# Autodesk Inventor assembly: BREEZE-S02
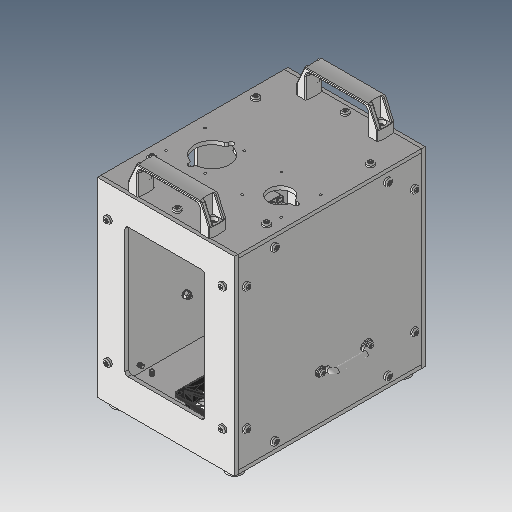
[picture p0: Inventor's stored thumbnail of the model, 512x512]
Saved by Autodesk Inventor 2020 (Build 240168000, 168)
## iProperties
Created: 2020-04-12
Part Number: BREEZE-S02
Document SubType Name: Assembly
Designer: John K
Description: PANEL ASSEMBLY
Author: John K
## Documents named in this file (22)
- C:\GrabCAD\MTL Ventilator Design\BREEZE\Subassemblies\BREEZE-S02.iam
- C:\GrabCAD\MTL Ventilator Design\BREEZE\Manufactured Parts\BREEZE-M05.ipt
- C:\GrabCAD\MTL Ventilator Design\BREEZE\Manufactured Parts\BREEZE-M10.ipt
- C:\GrabCAD\MTL Ventilator Design\BREEZE\Manufactured Parts\BREEZE-M06.ipt
- C:\GrabCAD\MTL Ventilator Design\BREEZE\Manufactured Parts\BREEZE-M07.ipt
- C:\GrabCAD\MTL Ventilator Design\BREEZE\Manufactured Parts\BREEZE-M08.ipt
- C:\GrabCAD\MTL Ventilator Design\BREEZE\Manufactured Parts\BREEZE-M09.ipt
- C:\GrabCAD\MTL Ventilator Design\BREEZE\Commercial Parts\McMaster\M5x10mm Nylon Screw.ipt
- C:\GrabCAD\MTL Ventilator Design\BREEZE\Commercial Parts\McMaster\Foot.ipt
- C:\GrabCAD\MTL Ventilator Design\BREEZE\Commercial Parts\McMaster\M4x16mm Nylon Screw.ipt
- C:\GrabCAD\MTL Ventilator Design\BREEZE\Commercial Parts\McMaster\M4 Nylon Washer.ipt
- C:\GrabCAD\MTL Ventilator Design\BREEZE\Commercial Parts\McMaster\M4 Locknut.ipt
- C:\GrabCAD\MTL Ventilator Design\BREEZE\Commercial Parts\McMaster\Handle.ipt
- C:\GrabCAD\MTL Ventilator Design\BREEZE\Commercial Parts\McMaster\M5x16mm Nylon Screw.ipt
- C:\GrabCAD\MTL Ventilator Design\BREEZE\Commercial Parts\McMaster\Webbing Guide.ipt
- C:\GrabCAD\MTL Ventilator Design\BREEZE\Commercial Parts\Electronics\Toggle Switch.ipt
- C:\GrabCAD\MTL Ventilator Design\BREEZE\Commercial Parts\Electronics\Switch Cover.ipt
- C:\GrabCAD\MTL Ventilator Design\BREEZE\Commercial Parts\Electronics\Power Connector.ipt
- C:\GrabCAD\MTL Ventilator Design\BREEZE\Commercial Parts\McMaster\M3 Nylon Washer.ipt
- C:\GrabCAD\MTL Ventilator Design\BREEZE\Commercial Parts\McMaster\M3 Locknut.ipt
- C:\GrabCAD\MTL Ventilator Design\BREEZE\Commercial Parts\McMaster\M3x16mm Nylon Screw.ipt
- C:\GrabCAD\MTL Ventilator Design\BREEZE\Commercial Parts\Electronics\Chassis Fan.ipt
## Components (103 placed, 21 different names)
1. BREEZE-M05:1 — Mate:1, Flush:1, Flush:2, Flush:3, Symmetry:1, Mate:4, Insert:23, Insert:24, Insert:25, Insert:26, Insert:27, Insert:28, Insert:40, Insert:41, Insert:42, Insert:43, Insert:48, Insert:49, Insert:50, Insert:51, Mate:16, Mate:17, Mate:18, Insert:92, Insert:93, Insert:94, Insert:95
2. BREEZE-M06:1 — Flush:4, Mate:2, Flush:5, Flush:6, Mate:3, Insert:1, Insert:2, Insert:3, Insert:4
3. BREEZE-M07:1 — Flush:6, Mate:3, Mate:4, Mate:5, Flush:7, Insert:5, Insert:6, Insert:7, Insert:8, Insert:9, Insert:10, Insert:11, Insert:29, Insert:65, Mate:12, Insert:70, Insert:71
4. BREEZE-M08:1 — Flush:7, Flush:8, Mate:6, Mate:8, Flush:9, Insert:12, Insert:13, Insert:14, Insert:15, Insert:37, Insert:38, Insert:39, Angle:1, Angle:2
5. BREEZE-M09:1 — Mate:7, Mate:8, Flush:9, Insert:16, Insert:17, Insert:18, Insert:19, Insert:20, Insert:21, Insert:22, Insert:36, Insert:62, Mate:11, Insert:68, Insert:69, Insert:76, Insert:77, Mate:13, Mate:14, Mate:15, Insert:78, Insert:79
6. BREEZE-M10:1 — Flush:2, Flush:3, Symmetry:1, Flush:4, Mate:2, Flush:5, Mate:5, Flush:8, Mate:6, Mate:7, Insert:30, Insert:31, Insert:32, Insert:33, Insert:34, Insert:35, Insert:56, Insert:57, Mate:9, Mate:10
7. Foot:1 — Insert:40
8. Foot:2 — Insert:41
9. Foot:3 — Insert:42
10. Foot:4 — Insert:43
11. Handle:1 — Insert:56, Mate:9
12. Handle:2 — Insert:57, Mate:10
13. Webbing Guide:1 — Insert:62, Mate:11, Insert:63, Insert:64
14. Webbing Guide:2 — Insert:65, Mate:12, Insert:66, Insert:67
15. Power Connector:1 — Mate:13, Mate:14, Mate:15, Insert:82, Insert:83
16. Toggle Switch:1 — Insert:76, Angle:1
17. Switch Cover:1 — Insert:77, Angle:2
18. Chassis Fan:1 — Mate:16, Mate:17, Mate:18, Insert:84, Insert:85, Insert:86, Insert:87
19. M4 Nylon Washer:9 — Insert:84, Insert:91
20. M4 Nylon Washer:10 — Insert:85, Insert:90
21. M4 Nylon Washer:11 — Insert:86, Insert:88
22. M4 Nylon Washer:12 — Insert:87, Insert:89
23. M4 Locknut:9 — Insert:88
24. M4 Locknut:10 — Insert:89
25. M4 Locknut:11 — Insert:90
26. M4 Locknut:12 — Insert:91
27. M4x16mm Nylon Screw:9 — Insert:92
28. M4x16mm Nylon Screw:10 — Insert:93
29. M4x16mm Nylon Screw:11 — Insert:94
30. M4x16mm Nylon Screw:12 — Insert:95
31. M3 Nylon Washer:1 — Insert:78, Insert:80
32. M3 Nylon Washer:2 — Insert:79, Insert:81
33. M3 Locknut:1 — Insert:80
34. M3 Locknut:2 — Insert:81
35. M3x16mm Nylon Screw:1 — Insert:82
36. M3x16mm Nylon Screw:2 — Insert:83
37. M4x16mm Nylon Screw:7 — Insert:66
38. M4x16mm Nylon Screw:8 — Insert:67
39. M4 Nylon Washer:5 — Insert:68, Insert:72
40. M4 Nylon Washer:6 — Insert:69, Insert:73
41. M4 Nylon Washer:7 — Insert:70, Insert:74
42. M4 Nylon Washer:8 — Insert:71, Insert:75
43. M4 Locknut:5 — Insert:72
44. M4 Locknut:6 — Insert:73
45. M4 Locknut:7 — Insert:74
46. M4 Locknut:8 — Insert:75
47. M4x16mm Nylon Screw:5 — Insert:63
48. M4x16mm Nylon Screw:6 — Insert:64
49. M5x16mm Nylon Screw:1
50. M5x16mm Nylon Screw:2
51. M5x16mm Nylon Screw:4
52. M5x16mm Nylon Screw:3
53. M4x16mm Nylon Screw:1
54. M4x16mm Nylon Screw:2
55. M4x16mm Nylon Screw:3
56. M4x16mm Nylon Screw:4
57. M4 Nylon Washer:1 — Insert:48, Insert:52
58. M4 Nylon Washer:2 — Insert:49, Insert:53
59. M4 Nylon Washer:3 — Insert:50, Insert:54
60. M4 Nylon Washer:4 — Insert:51, Insert:55
61. M4 Locknut:1 — Insert:52
62. M4 Locknut:2 — Insert:53
63. M4 Locknut:3 — Insert:54
64. M4 Locknut:4 — Insert:55
65. M5x10mm Nylon Screw:1 — Insert:1
66. M5x10mm Nylon Screw:2 — Insert:2
67. M5x10mm Nylon Screw:3 — Insert:3
68. M5x10mm Nylon Screw:4 — Insert:4
69. M5x10mm Nylon Screw:5 — Insert:5
70. M5x10mm Nylon Screw:6 — Insert:6
71. M5x10mm Nylon Screw:7 — Insert:7
72. M5x10mm Nylon Screw:8 — Insert:8
73. M5x10mm Nylon Screw:9 — Insert:9
74. M5x10mm Nylon Screw:10 — Insert:10
75. M5x10mm Nylon Screw:11 — Insert:11
76. M5x10mm Nylon Screw:12 — Insert:12
77. M5x10mm Nylon Screw:13 — Insert:13
78. M5x10mm Nylon Screw:14 — Insert:14
79. M5x10mm Nylon Screw:15 — Insert:15
80. M5x10mm Nylon Screw:16 — Insert:16
81. M5x10mm Nylon Screw:17 — Insert:17
82. M5x10mm Nylon Screw:18 — Insert:18
83. M5x10mm Nylon Screw:19 — Insert:19
84. M5x10mm Nylon Screw:20 — Insert:20
85. M5x10mm Nylon Screw:21 — Insert:21
86. M5x10mm Nylon Screw:22 — Insert:22
87. M5x10mm Nylon Screw:23 — Insert:23
88. M5x10mm Nylon Screw:24 — Insert:24
89. M5x10mm Nylon Screw:25 — Insert:25
90. M5x10mm Nylon Screw:26 — Insert:26
91. M5x10mm Nylon Screw:27 — Insert:27
92. M5x10mm Nylon Screw:28 — Insert:28
93. M5x10mm Nylon Screw:29 — Insert:29
94. M5x10mm Nylon Screw:30 — Insert:30
95. M5x10mm Nylon Screw:31 — Insert:31
96. M5x10mm Nylon Screw:32 — Insert:32
97. M5x10mm Nylon Screw:33 — Insert:33
98. M5x10mm Nylon Screw:34 — Insert:34
99. M5x10mm Nylon Screw:35 — Insert:35
100. M5x10mm Nylon Screw:36 — Insert:36
101. M5x10mm Nylon Screw:37 — Insert:37
102. M5x10mm Nylon Screw:38 — Insert:38
103. M5x10mm Nylon Screw:39 — Insert:39
## Relationships (125: Insert 95, Mate 18, Flush 9, Angle 2, Symmetry 1)
- Mate:1: BREEZE-M05:1
- Flush:1: BREEZE-M05:1
- Flush:2: BREEZE-M05:1 ↔ BREEZE-M10:1
- Flush:3: BREEZE-M05:1 ↔ BREEZE-M10:1
- Symmetry:1: BREEZE-M05:1 ↔ BREEZE-M10:1
- Flush:4: BREEZE-M06:1 ↔ BREEZE-M10:1
- Mate:2: BREEZE-M06:1 ↔ BREEZE-M10:1
- Flush:5: BREEZE-M06:1 ↔ BREEZE-M10:1
- Flush:6: BREEZE-M06:1 ↔ BREEZE-M07:1
- Mate:3: BREEZE-M06:1 ↔ BREEZE-M07:1
- Mate:4: BREEZE-M05:1 ↔ BREEZE-M07:1
- Mate:5: BREEZE-M07:1 ↔ BREEZE-M10:1
- Flush:7: BREEZE-M07:1 ↔ BREEZE-M08:1
- Flush:8: BREEZE-M08:1 ↔ BREEZE-M10:1
- Mate:6: BREEZE-M08:1 ↔ BREEZE-M10:1
- Mate:7: BREEZE-M09:1 ↔ BREEZE-M10:1
- Mate:8: BREEZE-M08:1 ↔ BREEZE-M09:1
- Flush:9: BREEZE-M08:1 ↔ BREEZE-M09:1
- Insert:1: BREEZE-M06:1 ↔ M5x10mm Nylon Screw:1
- Insert:2: BREEZE-M06:1 ↔ M5x10mm Nylon Screw:2
- Insert:3: BREEZE-M06:1 ↔ M5x10mm Nylon Screw:3
- Insert:4: BREEZE-M06:1 ↔ M5x10mm Nylon Screw:4
- Insert:5: BREEZE-M07:1 ↔ M5x10mm Nylon Screw:5
- Insert:6: BREEZE-M07:1 ↔ M5x10mm Nylon Screw:6
- Insert:7: BREEZE-M07:1 ↔ M5x10mm Nylon Screw:7
- Insert:8: BREEZE-M07:1 ↔ M5x10mm Nylon Screw:8
- Insert:9: BREEZE-M07:1 ↔ M5x10mm Nylon Screw:9
- Insert:10: BREEZE-M07:1 ↔ M5x10mm Nylon Screw:10
- Insert:11: BREEZE-M07:1 ↔ M5x10mm Nylon Screw:11
- Insert:12: BREEZE-M08:1 ↔ M5x10mm Nylon Screw:12
- Insert:13: BREEZE-M08:1 ↔ M5x10mm Nylon Screw:13
- Insert:14: BREEZE-M08:1 ↔ M5x10mm Nylon Screw:14
- Insert:15: BREEZE-M08:1 ↔ M5x10mm Nylon Screw:15
- Insert:16: BREEZE-M09:1 ↔ M5x10mm Nylon Screw:16
- Insert:17: BREEZE-M09:1 ↔ M5x10mm Nylon Screw:17
- Insert:18: BREEZE-M09:1 ↔ M5x10mm Nylon Screw:18
- Insert:19: BREEZE-M09:1 ↔ M5x10mm Nylon Screw:19
- Insert:20: BREEZE-M09:1 ↔ M5x10mm Nylon Screw:20
- Insert:21: BREEZE-M09:1 ↔ M5x10mm Nylon Screw:21
- Insert:22: BREEZE-M09:1 ↔ M5x10mm Nylon Screw:22
- Insert:23: BREEZE-M05:1 ↔ M5x10mm Nylon Screw:23
- Insert:24: BREEZE-M05:1 ↔ M5x10mm Nylon Screw:24
- Insert:25: BREEZE-M05:1 ↔ M5x10mm Nylon Screw:25
- Insert:26: BREEZE-M05:1 ↔ M5x10mm Nylon Screw:26
- Insert:27: BREEZE-M05:1 ↔ M5x10mm Nylon Screw:27
- Insert:28: BREEZE-M05:1 ↔ M5x10mm Nylon Screw:28
- Insert:29: BREEZE-M07:1 ↔ M5x10mm Nylon Screw:29
- Insert:30: BREEZE-M10:1 ↔ M5x10mm Nylon Screw:30
- Insert:31: BREEZE-M10:1 ↔ M5x10mm Nylon Screw:31
- Insert:32: BREEZE-M10:1 ↔ M5x10mm Nylon Screw:32
- Insert:33: BREEZE-M10:1 ↔ M5x10mm Nylon Screw:33
- Insert:34: BREEZE-M10:1 ↔ M5x10mm Nylon Screw:34
- Insert:35: BREEZE-M10:1 ↔ M5x10mm Nylon Screw:35
- Insert:36: BREEZE-M09:1 ↔ M5x10mm Nylon Screw:36
- Insert:37: BREEZE-M08:1 ↔ M5x10mm Nylon Screw:37
- Insert:38: BREEZE-M08:1 ↔ M5x10mm Nylon Screw:38
- Insert:39: BREEZE-M08:1 ↔ M5x10mm Nylon Screw:39
- Insert:40: BREEZE-M05:1 ↔ Foot:1
- Insert:41: BREEZE-M05:1 ↔ Foot:2
- Insert:42: BREEZE-M05:1 ↔ Foot:3
- Insert:43: BREEZE-M05:1 ↔ Foot:4
- [Insert]: Foot:4 ↔ M4x16mm Nylon Screw:1
- [Insert]: Foot:1 ↔ M4x16mm Nylon Screw:2
- [Insert]: Foot:2 ↔ M4x16mm Nylon Screw:3
- [Insert]: Foot:3 ↔ M4x16mm Nylon Screw:4
- Insert:48: BREEZE-M05:1 ↔ M4 Nylon Washer:1
- Insert:49: BREEZE-M05:1 ↔ M4 Nylon Washer:2
- Insert:50: BREEZE-M05:1 ↔ M4 Nylon Washer:3
- Insert:51: BREEZE-M05:1 ↔ M4 Nylon Washer:4
- Insert:52: M4 Nylon Washer:1 ↔ M4 Locknut:1
- Insert:53: M4 Nylon Washer:2 ↔ M4 Locknut:2
- Insert:54: M4 Nylon Washer:3 ↔ M4 Locknut:3
- Insert:55: M4 Nylon Washer:4 ↔ M4 Locknut:4
- Insert:56: BREEZE-M10:1 ↔ Handle:1
- Insert:57: BREEZE-M10:1 ↔ Handle:2
- Mate:9: BREEZE-M10:1 ↔ Handle:1
- Mate:10: BREEZE-M10:1 ↔ Handle:2
- [Insert]: Handle:2 ↔ M5x16mm Nylon Screw:1
- [Insert]: Handle:2 ↔ M5x16mm Nylon Screw:2
- [Insert]: Handle:1 ↔ M5x16mm Nylon Screw:4
- [Insert]: Handle:1 ↔ M5x16mm Nylon Screw:3
- Insert:62: BREEZE-M09:1 ↔ Webbing Guide:1
- Mate:11: BREEZE-M09:1 ↔ Webbing Guide:1
- Insert:63: Webbing Guide:1 ↔ M4x16mm Nylon Screw:5
- Insert:64: Webbing Guide:1 ↔ M4x16mm Nylon Screw:6
- Insert:65: BREEZE-M07:1 ↔ Webbing Guide:2
- Mate:12: BREEZE-M07:1 ↔ Webbing Guide:2
- Insert:66: Webbing Guide:2 ↔ M4x16mm Nylon Screw:7
- Insert:67: Webbing Guide:2 ↔ M4x16mm Nylon Screw:8
- Insert:68: BREEZE-M09:1 ↔ M4 Nylon Washer:5
- Insert:69: BREEZE-M09:1 ↔ M4 Nylon Washer:6
- Insert:70: BREEZE-M07:1 ↔ M4 Nylon Washer:7
- Insert:71: BREEZE-M07:1 ↔ M4 Nylon Washer:8
- Insert:72: M4 Nylon Washer:5 ↔ M4 Locknut:5
- Insert:73: M4 Nylon Washer:6 ↔ M4 Locknut:6
- Insert:74: M4 Nylon Washer:7 ↔ M4 Locknut:7
- Insert:75: M4 Nylon Washer:8 ↔ M4 Locknut:8
- Insert:76: BREEZE-M09:1 ↔ Toggle Switch:1
- Angle:1 (0 deg): BREEZE-M08:1 ↔ Toggle Switch:1
- Insert:77: BREEZE-M09:1 ↔ Switch Cover:1
- Angle:2 (0 deg): BREEZE-M08:1 ↔ Switch Cover:1
- Mate:13: BREEZE-M09:1 ↔ Power Connector:1
- Mate:14: BREEZE-M09:1 ↔ Power Connector:1
- Mate:15: BREEZE-M09:1 ↔ Power Connector:1
- Insert:78: BREEZE-M09:1 ↔ M3 Nylon Washer:1
- Insert:79: BREEZE-M09:1 ↔ M3 Nylon Washer:2
- Insert:80: M3 Nylon Washer:1 ↔ M3 Locknut:1
- Insert:81: M3 Nylon Washer:2 ↔ M3 Locknut:2
- Insert:82 (-0.635 mm): Power Connector:1 ↔ M3x16mm Nylon Screw:1
- Insert:83 (-0.635 mm): Power Connector:1 ↔ M3x16mm Nylon Screw:2
- Mate:16: BREEZE-M05:1 ↔ Chassis Fan:1
- Mate:17: BREEZE-M05:1 ↔ Chassis Fan:1
- Mate:18: BREEZE-M05:1 ↔ Chassis Fan:1
- Insert:84: Chassis Fan:1 ↔ M4 Nylon Washer:9
- Insert:85: Chassis Fan:1 ↔ M4 Nylon Washer:10
- Insert:86: Chassis Fan:1 ↔ M4 Nylon Washer:11
- Insert:87: Chassis Fan:1 ↔ M4 Nylon Washer:12
- Insert:88: M4 Nylon Washer:11 ↔ M4 Locknut:9
- Insert:89: M4 Nylon Washer:12 ↔ M4 Locknut:10
- Insert:90: M4 Nylon Washer:10 ↔ M4 Locknut:11
- Insert:91: M4 Nylon Washer:9 ↔ M4 Locknut:12
- Insert:92: BREEZE-M05:1 ↔ M4x16mm Nylon Screw:9
- Insert:93: BREEZE-M05:1 ↔ M4x16mm Nylon Screw:10
- Insert:94: BREEZE-M05:1 ↔ M4x16mm Nylon Screw:11
- Insert:95: BREEZE-M05:1 ↔ M4x16mm Nylon Screw:12
